# Autodesk Inventor assembly: ax-12a
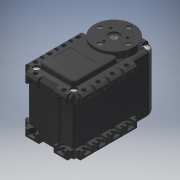
[picture p0: Inventor's stored thumbnail of the model, 180x180]
Saved by Autodesk Inventor 2019 (Build 230136000, 136)
## iProperties
Created: 2019-08-05
Part Number: ax-12a
Material: Типовые
Document SubType Name: Assembly
Designer: Петров Иван
Author: Петров Иван
## Documents named in this file (3)
- E:\IVAN\Kvantoriada2019\optimal_gripper\hardware\Стандартные изделия\Сервомотор Dynamixel AX-12A\ax-12a.iam
- E:\IVAN\Kvantoriada2019\optimal_gripper\hardware\Стандартные изделия\Сервомотор Dynamixel AX-12A\AX-12A_body.ipt
- E:\IVAN\Kvantoriada2019\optimal_gripper\hardware\Стандартные изделия\Сервомотор Dynamixel AX-12A\AX-12A_wheel.ipt
## Components (2 placed, 2 different names)
1. AX-12A_body:1 — Совмещение:1, Совмещение:2
2. AX-12A_wheel:1 — Совмещение:1, Совмещение:2
## Relationships (2: Mate 2)
- Совмещение:1 [Mate]: AX-12A_body:1 ↔ AX-12A_wheel:1
- Совмещение:2 [Mate]: AX-12A_body:1 ↔ AX-12A_wheel:1
